# Autodesk Inventor assembly: Blade set
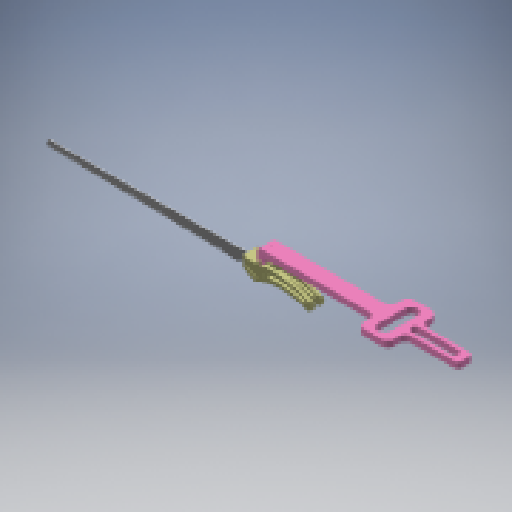
[picture p0: Inventor's stored thumbnail of the model, 512x512]
Saved by Autodesk Inventor 2024.1 (Build 281209000, 209)
## iProperties
Created: 2008-07-14
Part Number: Blade set
Document SubType Name: Assembly
Designer: tangg
Mass: 233.304 g
Surface Area: 206.898 cm^2
Volume: 29.7477 cm^3
Density: 7.84277 g/cm^3
Author: tangg
## Documents named in this file (4)
- D:\Descargas\Dynamic Simulation 1 and 2\Dynamic Simulation 1 and 2\Blade set.iam
- D:\Descargas\Dynamic Simulation 1 and 2\Dynamic Simulation 1 and 2\Blade clamp.ipt
- D:\Descargas\Dynamic Simulation 1 and 2\Dynamic Simulation 1 and 2\Saw blade.ipt
- D:\Descargas\Dynamic Simulation 1 and 2\Dynamic Simulation 1 and 2\Scottish Yoke.ipt
## Components (3 placed, 3 different names)
1. Scottish Yoke:1 — Mate:1, Flush:1
2. Blade clamp:1 — Mate:1, Flush:1, Mate:2, Mate:4
3. Saw blade:1 — Mate:2, Mate:4
## Relationships (5: Mate 4, Flush 1)
- Mate:1: Scottish Yoke:1 ↔ Blade clamp:1
- Flush:1: Scottish Yoke:1 ↔ Blade clamp:1
- [Mate]: Blade clamp:1 ↔ Saw blade:1
- Mate:2: Blade clamp:1 ↔ Saw blade:1
- Mate:4: Blade clamp:1 ↔ Saw blade:1
